# Autodesk Inventor assembly: Encoder_Mount3
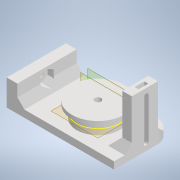
[picture p0: Inventor's stored thumbnail of the model, 180x180]
Saved by Autodesk Inventor 2022 (Build 260153000, 153)
## iProperties
Created: 2024-04-30
Part Number: Encoder_Mount3
Document SubType Name: Assembly
Designer: Gotham City
Author: Gotham City
## Documents named in this file (3)
- E:\inkjet-printer\cad\Encoder_Mount3.iam
- E:\inkjet-printer\cad\Encoder_Mount3_Wheel.ipt
- E:\inkjet-printer\cad\Encoder_Mount3_Base.ipt
## Components (2 placed, 2 different names)
1. Encoder_Mount3_Wheel:1 — Flush:1
2. Encoder_Mount3_Base:1 — Flush:1
## Relationships (1: Flush 1)
- Flush:1: Encoder_Mount3_Wheel:1 ↔ Encoder_Mount3_Base:1
